# Autodesk Inventor assembly: P&P Chocoperator Final Assembly
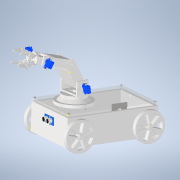
[picture p0: Inventor's stored thumbnail of the model, 180x180]
Saved by Autodesk Inventor 2022 (Build 260153000, 153)
## iProperties
Created: 2021-07-27
Part Number: P&P Chocoperator Final Assembly
Document SubType Name: Assembly
Designer: USER
Author: USER
## Documents named in this file (3)
- F:\BVB\robotic arm\P&P Chocoperator Final Assembly.iam
- F:\BVB\robotic arm\Base Assembly 1.iam
- F:\BVB\robotic arm\Robotic Arm Assembly 1(new).iam
## Components (2 placed, 2 different names)
1. Base Assembly 1:1 [sub-assembly] — Mate:1, Mate:2
2. Robotic Arm Assembly 1(new):1 [sub-assembly] — Mate:1, Mate:2
## Relationships (2: Mate 2)
- Mate:1: Base Assembly 1:1 ↔ Robotic Arm Assembly 1(new):1
- Mate:2: Base Assembly 1:1 ↔ Robotic Arm Assembly 1(new):1
